# Autodesk Inventor assembly: Sides
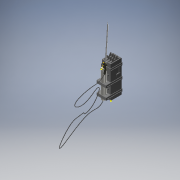
[picture p0: Inventor's stored thumbnail of the model, 180x180]
Saved by Autodesk Inventor 2021 (Build 250183000, 183)
## iProperties
Created: 2021-05-30
Part Number: Sides
Document SubType Name: Assembly
Designer: AHUJA
Author: AHUJA
## Documents named in this file (6)
- F:\Files\ODM GEAR IPT\My worl\Sides.iam
- F:\Files\ODM GEAR IPT\My worl\Gas.iam
- F:\Files\ODM GEAR IPT\My worl\Gas + Blade Holder.ipt
- F:\Files\ODM GEAR IPT\My worl\Spare Blade (In Blade Holder).ipt
- F:\Files\ODM GEAR IPT\My worl\Gas Wire.ipt
- F:\Files\ODM GEAR IPT\My worl\Shingeki no Kyojin Blade.ipt
## Components (8 placed, 5 different names)
1. Gas:1 [sub-assembly] — Mate:1, Flush:1, Mate:10
2. Gas + Blade Holder:1 — Mate:1, Flush:1, Mate:2, Mate:3, Mate:4, Mate:5, Mate:6, Mate:7, Mate:8, Mate:9
3. Spare Blade (In Blade Holder):1 — Mate:2, Mate:3, Flush:2
4. Spare Blade (In Blade Holder):2 — Mate:4, Mate:5, Flush:2, Flush:3
5. Spare Blade (In Blade Holder):3 — Mate:6, Mate:7, Flush:3, Flush:4
6. Spare Blade (In Blade Holder):4 — Mate:8, Mate:9, Flush:4
7. Gas Wire:1 — Mate:10, Mate:11
8. Shingeki no Kyojin Blade:1 — Mate:11
## Relationships (15: Mate 11, Flush 4)
- Mate:1: Gas:1 ↔ Gas + Blade Holder:1
- Flush:1: Gas:1 ↔ Gas + Blade Holder:1
- Mate:2: Gas + Blade Holder:1 ↔ Spare Blade (In Blade Holder):1
- Mate:3 (15 mm): Gas + Blade Holder:1 ↔ Spare Blade (In Blade Holder):1
- Mate:4: Gas + Blade Holder:1 ↔ Spare Blade (In Blade Holder):2
- Mate:5 (15 mm): Gas + Blade Holder:1 ↔ Spare Blade (In Blade Holder):2
- Mate:6: Gas + Blade Holder:1 ↔ Spare Blade (In Blade Holder):3
- Mate:7 (15 mm): Gas + Blade Holder:1 ↔ Spare Blade (In Blade Holder):3
- Mate:8: Gas + Blade Holder:1 ↔ Spare Blade (In Blade Holder):4
- Mate:9 (15 mm): Gas + Blade Holder:1 ↔ Spare Blade (In Blade Holder):4
- Flush:2: Spare Blade (In Blade Holder):1 ↔ Spare Blade (In Blade Holder):2
- Flush:3: Spare Blade (In Blade Holder):2 ↔ Spare Blade (In Blade Holder):3
- Flush:4: Spare Blade (In Blade Holder):3 ↔ Spare Blade (In Blade Holder):4
- Mate:10: Gas:1 ↔ Gas Wire:1
- Mate:11: Gas Wire:1 ↔ Shingeki no Kyojin Blade:1
